# Autodesk Inventor assembly: Wheel Assembly
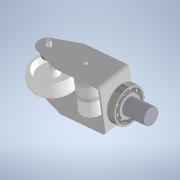
[picture p0: Inventor's stored thumbnail of the model, 180x180]
Saved by Autodesk Inventor 2020 (Build 240168000, 168)
## iProperties
Created: 2022-07-01
Part Number: Wheel Assembly
Document SubType Name: Assembly
Designer: karimi2
Author: karimi2
## Documents named in this file (8)
- C:\Users\karimi2\Documents\PROJECT\Wheel Assembly.iam
- C:\Users\karimi2\Documents\PROJECT\New frame.ipt
- C:\Users\karimi2\Documents\PROJECT\GearedDCmotor.ipt
- C:\Users\karimi2\Documents\PROJECT\wheelshaftGenerated.ipt
- C:\Users\karimi2\Documents\PROJECT\casterwheel.ipt
- C:\Users\karimi2\Documents\PROJECT\Wheel Assembly\Design Accelerator\Synchronous Belts Transmission1.iam
- C:\Users\karimi2\Documents\PROJECT\topshaft.ipt
- C:\Users\karimi2\Documents\PROJECT\BearingGenerated.iam
## Components (7 placed, 7 different names)
1. New frame:1 — Mate:1, Mate:2, Mate:3, Mate:4, Mate:6, Mate:8, Rigid:1, Flush:1
2. GearedDCmotor:1 — Mate:1, Mate:2, Mate:7
3. Shaft:1 — Mate:3, Mate:4, Mate:5, Mate:9
4. casterwheel:1 — Mate:5, Mate:6
5. Synchronous Belts Transmission:1 [sub-assembly] — Mate:7, Mate:8, Mate:9
6. topshaft:1 — Rigid:1, Mate:10
7. Bearing:1 [sub-assembly] — Mate:10, Flush:1
## Relationships (12: Mate 10, WeldJoint 1, Flush 1)
- Mate:1: New frame:1 ↔ GearedDCmotor:1
- Mate:2 (-40 mm): New frame:1 ↔ GearedDCmotor:1
- Mate:3: New frame:1 ↔ Shaft:1
- Mate:4 (-9 mm): New frame:1 ↔ Shaft:1
- Mate:5: Shaft:1 ↔ casterwheel:1
- Mate:6 (10 mm): New frame:1 ↔ casterwheel:1
- Mate:7: GearedDCmotor:1 ↔ Synchronous Belts Transmission:1
- Mate:8: New frame:1 ↔ Synchronous Belts Transmission:1
- Mate:9: Shaft:1 ↔ Synchronous Belts Transmission:1
- Rigid:1 [WeldJoint]: New frame:1 ↔ topshaft:1
- Mate:10: topshaft:1 ↔ Bearing:1
- Flush:1 (-7 mm): New frame:1 ↔ Bearing:1
